# Autodesk Inventor assembly: AssemblyFinal
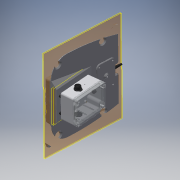
[picture p0: Inventor's stored thumbnail of the model, 180x180]
Saved by Autodesk Inventor 2019 (Build 230136000, 136)
## iProperties
Created: 2019-04-20
Part Number: AssemblyFinal
Document SubType Name: Assembly
Designer: lgnds
Author: lgnds
## Documents named in this file (10)
- C:\Users\CASE-SMALL2\Google Drive\Kandidatarbete Rescuerunner\Drive-by-wire\Design docummentation\Front Rail System\FrontPanelMount\AssemblyFinal.iam
- C:\Users\CASE-SMALL2\Google Drive\Kandidatarbete Rescuerunner\Drive-by-wire\Design docummentation\Front Rail System\FrontPanelMount\FrontPanelMountMeshFinal.ipt
- C:\Users\CASE-SMALL2\Google Drive\Kandidatarbete Rescuerunner\Drive-by-wire\Design docummentation\Front Rail System\FrontPanelMount\GPS_AND_RCU_MOUNT_V4.ipt
- C:\Users\CASE-SMALL2\Google Drive\Kandidatarbete Rescuerunner\Drive-by-wire\Design docummentation\Front Rail System\CAD_BOX_RCU\RCU_Assembly.iam
- C:\Users\CASE-SMALL2\Google Drive\Kandidatarbete Rescuerunner\Drive-by-wire\Design docummentation\Front Rail System\FrontPanelMount\GPS_Antenna.ipt
- C:\Users\CASE-SMALL2\Google Drive\Kandidatarbete Rescuerunner\Drive-by-wire\Design docummentation\Front Rail System\FrontPanelMount\GPS_Antenna_Fix.ipt
- C:\Users\CASE-SMALL2\Google Drive\Kandidatarbete Rescuerunner\Drive-by-wire\Design docummentation\Front Rail System\FrontPanelMount\HoleFill1.ipt
- C:\Users\CASE-SMALL2\Google Drive\Kandidatarbete Rescuerunner\Drive-by-wire\Design docummentation\Front Rail System\FrontPanelMount\HoleFill3.ipt
- C:\Users\CASE-SMALL2\Google Drive\Kandidatarbete Rescuerunner\Drive-by-wire\Design docummentation\Front Rail System\FrontPanelMount\HoleFill4.ipt
- C:\Users\CASE-SMALL2\Google Drive\Kandidatarbete Rescuerunner\Drive-by-wire\Design docummentation\Front Rail System\FrontPanelMount\HoleFill2.ipt
## Components (13 placed, 9 different names)
1. FrontPanelMountMeshFinal:1 — Mate:2, Mate:6, Flush:1
2. GPS_AND_RCU_MOUNT_V4:1 — Mate:2, Mate:3, Mate:4, Mate:5, Mate:6, Flush:1, Flush:2, Mate:7, Mate:8, Angle:1, Rotational:1, Rotational:2, Rotational:3, Rotational:4, Rotational:5, Rotational:6, Rigid:1, Rigid:2
3. RCU_Assembly:1 [sub-assembly] — Mate:3, Mate:4, Mate:5
4. GPS_Antenna:1 — Flush:2, Mate:7, Mate:8, Insert:1
5. GPS_Antenna_Fix:1 — Insert:1, Angle:1
6. HoleFill1:1 — Rotational:2
7. HoleFill1:2 — Rotational:1
8. HoleFill3:1 — Rotational:3
9. HoleFill3:2 — Rotational:4
10. HoleFill4:1 — Rotational:5
11. HoleFill4:2 — Rotational:6
12. HoleFill2:1 — Rigid:1
13. HoleFill2:2 — Rigid:2
## Relationships (19: Mate 7, RevoluteJoint 6, Flush 2, WeldJoint 2, Insert 1, Angle 1)
- Mate:2 (-2 mm): FrontPanelMountMeshFinal:1 ↔ GPS_AND_RCU_MOUNT_V4:1
- Mate:3: GPS_AND_RCU_MOUNT_V4:1 ↔ RCU_Assembly:1
- Mate:4: GPS_AND_RCU_MOUNT_V4:1 ↔ RCU_Assembly:1
- Mate:5: GPS_AND_RCU_MOUNT_V4:1 ↔ RCU_Assembly:1
- Mate:6 (-3 mm): FrontPanelMountMeshFinal:1 ↔ GPS_AND_RCU_MOUNT_V4:1
- Flush:1: FrontPanelMountMeshFinal:1 ↔ GPS_AND_RCU_MOUNT_V4:1
- Flush:2: GPS_AND_RCU_MOUNT_V4:1 ↔ GPS_Antenna:1
- Mate:7 (1 mm): GPS_AND_RCU_MOUNT_V4:1 ↔ GPS_Antenna:1
- Mate:8 (0.5 mm): GPS_AND_RCU_MOUNT_V4:1 ↔ GPS_Antenna:1
- Insert:1: GPS_Antenna:1 ↔ GPS_Antenna_Fix:1
- Angle:1 (0 deg): GPS_AND_RCU_MOUNT_V4:1 ↔ GPS_Antenna_Fix:1
- Rotational:1 [RevoluteJoint]: GPS_AND_RCU_MOUNT_V4:1 ↔ HoleFill1:2
- Rotational:2 [RevoluteJoint]: GPS_AND_RCU_MOUNT_V4:1 ↔ HoleFill1:1
- Rotational:3 [RevoluteJoint]: GPS_AND_RCU_MOUNT_V4:1 ↔ HoleFill3:1
- Rotational:4 [RevoluteJoint]: GPS_AND_RCU_MOUNT_V4:1 ↔ HoleFill3:2
- Rotational:5 [RevoluteJoint]: GPS_AND_RCU_MOUNT_V4:1 ↔ HoleFill4:1
- Rotational:6 [RevoluteJoint]: GPS_AND_RCU_MOUNT_V4:1 ↔ HoleFill4:2
- Rigid:1 [WeldJoint]: GPS_AND_RCU_MOUNT_V4:1 ↔ HoleFill2:1
- Rigid:2 [WeldJoint]: GPS_AND_RCU_MOUNT_V4:1 ↔ HoleFill2:2
